# Autodesk Inventor assembly: LaundryRobot_v01
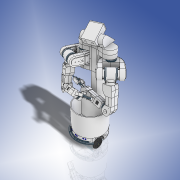
[picture p0: Inventor's stored thumbnail of the model, 180x180]
Saved by Autodesk Inventor 2017 SP1 (Build 210196100, 196)
## iProperties
Created: 2017-03-11
Part Number: LaundryRobot_v01
Document SubType Name: Assembly
Designer: zallen
Author: zallen
## Documents named in this file (6)
- C:\Users\Zach\Documents\GitHub\cr-laundry-robot\LaundryRobot_v01.iam
- C:\Users\Zach\Documents\GitHub\cr-laundry-robot\src\Base\Base.iam
- C:\Users\Zach\Documents\GitHub\cr-laundry-robot\src\Body\Body.iam
- C:\Users\Zach\Documents\GitHub\cr-laundry-robot\src\Head\Head.iam
- C:\Users\Zach\Documents\GitHub\cr-laundry-robot\src\Base 2\Base2.iam
- C:\Users\Zach\Documents\GitHub\cr-laundry-robot\src\Body 2\Body2.iam
## Components (6 placed, 5 different names)
1. Base:1 [sub-assembly] — Mate:1, Mate:2, Mate:4, Mate:5, Mate:6
2. Body:1 [sub-assembly] — Mate:1, Mate:2, Mate:7, Mate:8, Mate:9
3. Head:1 [sub-assembly] — Mate:7, Mate:8, Mate:9
4. Base2:1 [sub-assembly] — Mate:11, Mate:12, Mate:13, Mate:14
5. Body2:1 [sub-assembly] — Mate:13, Mate:14, Mate:15, Mate:16, Mate:17
6. Head:2 [sub-assembly] — Mate:15, Mate:16, Mate:17
## Relationships (15: Mate 15)
- Mate:1: Base:1 ↔ Body:1
- Mate:2: Base:1 ↔ Body:1
- Mate:4: Base:1
- Mate:5: Base:1
- Mate:6: Base:1
- Mate:7: Body:1 ↔ Head:1
- Mate:8: Body:1 ↔ Head:1
- Mate:9: Body:1 ↔ Head:1
- Mate:11: Base2:1
- Mate:12: Base2:1
- Mate:13: Base2:1 ↔ Body2:1
- Mate:14: Base2:1 ↔ Body2:1
- Mate:15: Body2:1 ↔ Head:2
- Mate:16: Body2:1 ↔ Head:2
- Mate:17: Body2:1 ↔ Head:2
